# Autodesk Inventor assembly: Carousel Base Plate Assembly
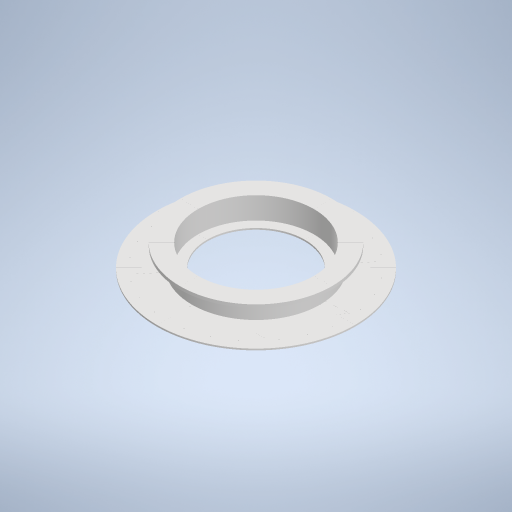
[picture p0: Inventor's stored thumbnail of the model, 512x512]
Saved by Autodesk Inventor 2023 (Build 270158000, 158)
## iProperties
Created: 2023-02-06
Part Number: Carousel Base Plate Assembly
Document SubType Name: Assembly
Designer: cheng
Author: cheng
## Documents named in this file (2)
- C:\Users\cheng\Desktop\4th Year Project\Inventor\Ninth Assembly\Carousel Base Plate Assembly.iam
- C:\Users\cheng\Desktop\4th Year Project\Inventor\Ninth Assembly\Carousel Base Plate v2.ipt
## Components (8 placed, 1 different names)
1. Carousel Base Plate v2:1 — Mate:5, Mate:6, Flush:3, Mate:9, Flush:6, Mate:10
2. Carousel Base Plate v2:2 — Mate:9, Flush:6, Mate:10, Mate:11, Flush:7, Mate:12
3. Carousel Base Plate v2:3 — Mate:11, Flush:7, Mate:12, Mate:13, Flush:8, Mate:14
4. Carousel Base Plate v2:4 — Mate:13, Flush:8, Mate:14
5. Carousel Base Plate v2:5 — Mate:1, Flush:1, Mate:2, Mate:3, Flush:2, Mate:4
6. Carousel Base Plate v2:6 — Mate:3, Flush:2, Mate:4, Mate:7, Flush:4, Flush:5, Mate:8
7. Carousel Base Plate v2:7 — Mate:7, Flush:4, Flush:5, Mate:8
8. Carousel Base Plate v2:8 — Mate:1, Flush:1, Mate:2, Mate:5, Mate:6, Flush:3
## Relationships (22: Mate 14, Flush 8)
- Mate:1: Carousel Base Plate v2:5 ↔ Carousel Base Plate v2:8
- Flush:1: Carousel Base Plate v2:5 ↔ Carousel Base Plate v2:8
- Mate:2: Carousel Base Plate v2:5 ↔ Carousel Base Plate v2:8
- Mate:3: Carousel Base Plate v2:5 ↔ Carousel Base Plate v2:6
- Flush:2: Carousel Base Plate v2:5 ↔ Carousel Base Plate v2:6
- Mate:4: Carousel Base Plate v2:5 ↔ Carousel Base Plate v2:6
- Mate:5: Carousel Base Plate v2:1 ↔ Carousel Base Plate v2:8
- Mate:6: Carousel Base Plate v2:1 ↔ Carousel Base Plate v2:8
- Flush:3: Carousel Base Plate v2:1 ↔ Carousel Base Plate v2:8
- Mate:7: Carousel Base Plate v2:6 ↔ Carousel Base Plate v2:7
- Flush:4: Carousel Base Plate v2:6 ↔ Carousel Base Plate v2:7
- Flush:5: Carousel Base Plate v2:6 ↔ Carousel Base Plate v2:7
- Mate:8: Carousel Base Plate v2:6 ↔ Carousel Base Plate v2:7
- Mate:9: Carousel Base Plate v2:1 ↔ Carousel Base Plate v2:2
- Flush:6: Carousel Base Plate v2:1 ↔ Carousel Base Plate v2:2
- Mate:10: Carousel Base Plate v2:1 ↔ Carousel Base Plate v2:2
- Mate:11: Carousel Base Plate v2:2 ↔ Carousel Base Plate v2:3
- Flush:7: Carousel Base Plate v2:2 ↔ Carousel Base Plate v2:3
- Mate:12: Carousel Base Plate v2:2 ↔ Carousel Base Plate v2:3
- Mate:13: Carousel Base Plate v2:3 ↔ Carousel Base Plate v2:4
- Flush:8: Carousel Base Plate v2:3 ↔ Carousel Base Plate v2:4
- Mate:14: Carousel Base Plate v2:3 ↔ Carousel Base Plate v2:4
